# Autodesk Inventor assembly: gripper jaw
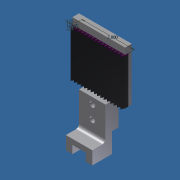
[picture p0: Inventor's stored thumbnail of the model, 180x180]
Saved by Autodesk Inventor 2012 (Build 160160000, 160)
## iProperties
Created: 2012-08-09
Part Number: gripper jaw
Document SubType Name: Assembly
Designer: Edward
Author: Edward
## Documents named in this file (4)
- C:\Users\Ed\Documents\masters\CAD\Gripper\gripper jaw.iam
- C:\Users\Ed\Documents\masters\CAD\Gripper\gripper jaw extension.ipt
- C:\Users\Ed\Documents\masters\CAD\Gripper\gripper jaw.ipt
- C:\Users\Ed\Documents\masters\CAD\Gripper\gripper pad.ipt
## Components (3 placed, 3 different names)
1. gripper jaw extension:1 — Mate:1, Flush:1, Mate:2, Insert:1, Insert:2
2. gripper jaw:1 — Insert:1, Insert:2
3. gripper pad:1 — Mate:1, Flush:1, Mate:2
## Relationships (5: Mate 2, Insert 2, Flush 1)
- Mate:1: gripper jaw extension:1 ↔ gripper pad:1
- Flush:1: gripper jaw extension:1 ↔ gripper pad:1
- Mate:2: gripper jaw extension:1 ↔ gripper pad:1
- Insert:1: gripper jaw extension:1 ↔ gripper jaw:1
- Insert:2: gripper jaw extension:1 ↔ gripper jaw:1
